# Autodesk Inventor assembly: Assembly_Opentrons_Imagingunit_v2
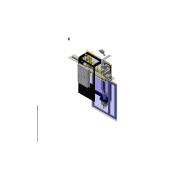
[picture p0: Inventor's stored thumbnail of the model, 180x180]
Saved by Autodesk Inventor 2019.4 (Build 234330000, 330)
## iProperties
Created: 2020-10-27
Part Number: Assembly_Opentrons_Imagingunit_v2
Document SubType Name: Assembly
Designer: diederichbenedict
Author: diederichbenedict
## Documents named in this file (14)
- C:\Users\diederichbenedict\Dropbox\Dokumente\Promotion\PROJECTS\OPENTRONS\INVENTOR\Assembly_Opentrons_Imagingunit_v2.iam
- C:\Users\diederichbenedict\Dropbox\Dokumente\Promotion\PROJECTS\OPENTRONS\INVENTOR\00_MTP_96-welplate.ipt
- C:\Users\diederichbenedict\Dropbox\Dokumente\Promotion\PROJECTS\OPENTRONS\INVENTOR\04_OPENTRONS_Microscope_wellplate_base.ipt
- C:\Users\diederichbenedict\Dropbox\Dokumente\Promotion\PROJECTS\OPENTRONS\INVENTOR\Assembly_opentrons_microscope_slide_y.iam
- C:\Users\diederichbenedict\Dropbox\Dokumente\Promotion\PROJECTS\OPENTRONS\INVENTOR\Assembly_opentrons_microscope_slide_y_base.iam
- C:\Users\diederichbenedict\Dropbox\Dokumente\Promotion\PROJECTS\OPENTRONS\INVENTOR\00_Endstop.ipt
- C:\Users\diederichbenedict\Dropbox\Dokumente\Promotion\PROJECTS\OPENTRONS\INVENTOR\09_Opentrons_Microscope_Baseplate.ipt
- C:\Users\diederichbenedict\Dropbox\Dokumente\Promotion\PROJECTS\OPENTRONS\INVENTOR\00_MGN12 LINEAR GUIDE RAIL, CONFIGURABLE.ipt
- C:\Users\diederichbenedict\Dropbox\Dokumente\Promotion\PROJECTS\OPENTRONS\INVENTOR\00_MGN12H, LINEAR GUIDE BLOCK.ipt
- C:\Users\diederichbenedict\Dropbox\Dokumente\Promotion\PROJECTS\OPENTRONS\INVENTOR\00_spindel_slide.ipt
- C:\Users\diederichbenedict\Dropbox\Dokumente\Promotion\PROJECTS\OPENTRONS\INVENTOR\00_Thorlabs_Rod_200mm.ipt
- C:\Users\diederichbenedict\Dropbox\Dokumente\Promotion\PROJECTS\OPENTRONS\INVENTOR\16_Opentrons_Microscope_Slide_Bearing.ipt
- C:\Users\diederichbenedict\Dropbox\Dokumente\Promotion\PROJECTS\OPENTRONS\INVENTOR\Assembly_Opentrons_Autofocus_v2.iam
- C:\Users\diederichbenedict\Dropbox\Dokumente\Promotion\PROJECTS\OPENTRONS\INVENTOR\OPENTRONS_Autofocus_clutch_Nema.ipt
## Components (14 placed, 13 different names)
1. 00_Endstop:1
2. Assembly_opentrons_microscope_slide_y_base:1 [sub-assembly] — Mate:18, Mate:23, Flush:5, Mate:32, Angle:1, Angle:2, Mate:34
3. 09_Opentrons_Microscope_Baseplate:1 — Flush:5
4. 00_spindel_slide:1 — Mate:18
5. 00_MGN12 LINEAR GUIDE RAIL, CONFIGURABLE:2 — Mate:23
6. 04_OPENTRONS_Microscope_wellplate_base:1
7. 00_Thorlabs_Rod_200mm:1
8. 16_Opentrons_Microscope_Slide_Bearing:1
9. OPENTRONS_Autofocus_clutch_Nema:1
10. 00_MTP_96-welplate:1
11. Assembly_Opentrons_Autofocus_v2:1 [sub-assembly] — Mate:33, Angle:2
12. Assembly_opentrons_microscope_slide_y:1 [sub-assembly] — Mate:32, Angle:1, Mate:33
13. 00_MGN12 LINEAR GUIDE RAIL, CONFIGURABLE:3 — Mate:34, Mate:35, Mate:36
14. 00_MGN12H, LINEAR GUIDE BLOCK:1 — Mate:35, Mate:36
## Relationships (10: Mate 7, Angle 2, Flush 1)
- Mate:18: Assembly_opentrons_microscope_slide_y_base:1 ↔ 00_spindel_slide:1
- Mate:23 (2 mm): Assembly_opentrons_microscope_slide_y_base:1 ↔ 00_MGN12 LINEAR GUIDE RAIL, CONFIGURABLE:2
- Flush:5: Assembly_opentrons_microscope_slide_y_base:1 ↔ 09_Opentrons_Microscope_Baseplate:1
- Mate:32: Assembly_opentrons_microscope_slide_y_base:1 ↔ Assembly_opentrons_microscope_slide_y:1
- Angle:1 (0 deg): Assembly_opentrons_microscope_slide_y_base:1 ↔ Assembly_opentrons_microscope_slide_y:1
- Mate:33: Assembly_Opentrons_Autofocus_v2:1 ↔ Assembly_opentrons_microscope_slide_y:1
- Angle:2 (0 deg): Assembly_opentrons_microscope_slide_y_base:1 ↔ Assembly_Opentrons_Autofocus_v2:1
- Mate:34: Assembly_opentrons_microscope_slide_y_base:1 ↔ 00_MGN12 LINEAR GUIDE RAIL, CONFIGURABLE:3
- Mate:35: 00_MGN12 LINEAR GUIDE RAIL, CONFIGURABLE:3 ↔ 00_MGN12H, LINEAR GUIDE BLOCK:1
- Mate:36: 00_MGN12 LINEAR GUIDE RAIL, CONFIGURABLE:3 ↔ 00_MGN12H, LINEAR GUIDE BLOCK:1
